# Autodesk Inventor assembly: rover-encoder-assembly
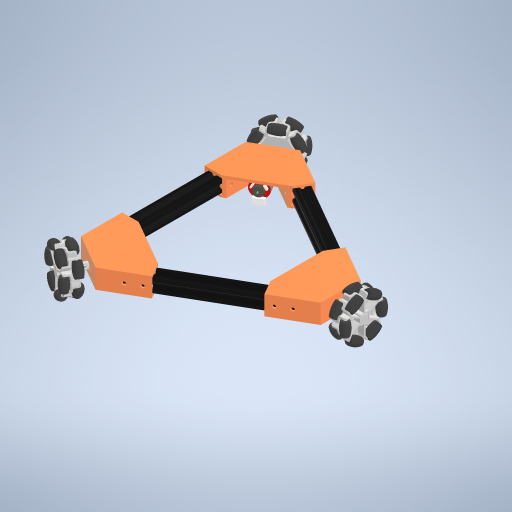
[picture p0: Inventor's stored thumbnail of the model, 512x512]
Saved by Autodesk Inventor 2024.2 (Build 282272000, 272)
## iProperties
Created: 2024-04-23
Part Number: rover-encoder-assembly
Document SubType Name: Assembly
Designer: Robin
Author: Robin
## Documents named in this file (6)
- C:\Users\Robin\OneDrive\Study\Current\Mechanical Design\Cad\fork-cad\rover-encoder-assembly.iam
- C:\Users\Robin\OneDrive\Study\Current\Mechanical Design\Cad\fork-cad\cornerBracket_Encoder.ipt
- C:\Users\Robin\OneDrive\Study\Current\Mechanical Design\Cad\fork-cad\2020aluminum_extrusion_black.ipt
- C:\Users\Robin\OneDrive\Study\Current\Mechanical Design\Cad\fork-cad\JGA25-370 DC12V350RPM\JGA25-370 DC12V350RPM.ipt
- C:\Users\Robin\OneDrive\Study\Current\Mechanical Design\Cad\fork-cad\wheel-assembly.iam
- C:\Users\Robin\OneDrive\Study\Current\Mechanical Design\Cad\fork-cad\holo-lock.ipt
## Components (15 placed, 5 different names)
1. cornerBracket_Encoder:1 — Mate:1, Mate:2, Mate:3, Mate:4, Mate:5, Mate:6, Mate:18, Mate:19, Mate:31
2. cornerBracket_Encoder:2 — Mate:10, Mate:11, Mate:12, Mate:13, Mate:14, Mate:15, Mate:17, Mate:20, Mate:33
3. cornerBracket_Encoder:3 — Mate:7, Mate:8, Mate:9, Mate:16, Mate:21, Mate:29
4. 2020aluminum_extrusion_black:1 — Mate:11, Mate:12, Mate:13
5. 2020aluminum_extrusion_black:2 — Mate:4, Mate:5, Mate:6, Mate:7, Mate:8, Mate:9
6. 2020aluminum_extrusion_black:3 — Mate:1, Mate:2, Mate:3, Mate:10, Mate:14, Mate:15
7. JGA25-370 DC12V350RPM:1 — Mate:17, Mate:20, Mate:32
8. JGA25-370 DC12V350RPM:2 — Mate:16, Mate:21, Mate:28
9. JGA25-370 DC12V350RPM:3 — Mate:18, Mate:19, Mate:30
10. wheel-assembly:1 [sub-assembly] — Mate:22, Mate:23, Flush:1
11. holo-lock:1 — Mate:22, Mate:23, Flush:1, Mate:32, Mate:33
12. wheel-assembly:4 [sub-assembly]
13. holo-lock:4 — Mate:30, Mate:31
14. wheel-assembly:5 [sub-assembly]
15. holo-lock:5 — Mate:28, Mate:29
## Relationships (36: Mate 33, Flush 3)
- Mate:1: cornerBracket_Encoder:1 ↔ 2020aluminum_extrusion_black:3
- Mate:2 (0.5 mm): cornerBracket_Encoder:1 ↔ 2020aluminum_extrusion_black:3
- Mate:3 (0.5 mm): cornerBracket_Encoder:1 ↔ 2020aluminum_extrusion_black:3
- Mate:4: cornerBracket_Encoder:1 ↔ 2020aluminum_extrusion_black:2
- Mate:5 (0.5 mm): cornerBracket_Encoder:1 ↔ 2020aluminum_extrusion_black:2
- Mate:6 (0.5 mm): cornerBracket_Encoder:1 ↔ 2020aluminum_extrusion_black:2
- Mate:7: cornerBracket_Encoder:3 ↔ 2020aluminum_extrusion_black:2
- Mate:8 (0.5 mm): cornerBracket_Encoder:3 ↔ 2020aluminum_extrusion_black:2
- Mate:9 (0.5 mm): cornerBracket_Encoder:3 ↔ 2020aluminum_extrusion_black:2
- Mate:10: cornerBracket_Encoder:2 ↔ 2020aluminum_extrusion_black:3
- Mate:11: cornerBracket_Encoder:2 ↔ 2020aluminum_extrusion_black:1
- Mate:12 (0.5 mm): cornerBracket_Encoder:2 ↔ 2020aluminum_extrusion_black:1
- Mate:13 (0.5 mm): cornerBracket_Encoder:2 ↔ 2020aluminum_extrusion_black:1
- Mate:14 (0.5 mm): cornerBracket_Encoder:2 ↔ 2020aluminum_extrusion_black:3
- Mate:15 (0.5 mm): cornerBracket_Encoder:2 ↔ 2020aluminum_extrusion_black:3
- Mate:16: cornerBracket_Encoder:3 ↔ JGA25-370 DC12V350RPM:2
- Mate:17: cornerBracket_Encoder:2 ↔ JGA25-370 DC12V350RPM:1
- Mate:18: cornerBracket_Encoder:1 ↔ JGA25-370 DC12V350RPM:3
- Mate:19: cornerBracket_Encoder:1 ↔ JGA25-370 DC12V350RPM:3
- Mate:20: cornerBracket_Encoder:2 ↔ JGA25-370 DC12V350RPM:1
- Mate:21: cornerBracket_Encoder:3 ↔ JGA25-370 DC12V350RPM:2
- Mate:22: wheel-assembly:1 ↔ holo-lock:1
- Mate:23: wheel-assembly:1 ↔ holo-lock:1
- Flush:1: wheel-assembly:1 ↔ holo-lock:1
- [Mate]: wheel-assembly:4 ↔ holo-lock:4
- [Mate]: wheel-assembly:4 ↔ holo-lock:4
- [Flush]: wheel-assembly:4 ↔ holo-lock:4
- [Mate]: wheel-assembly:5 ↔ holo-lock:5
- [Mate]: wheel-assembly:5 ↔ holo-lock:5
- [Flush]: wheel-assembly:5 ↔ holo-lock:5
- Mate:28: JGA25-370 DC12V350RPM:2 ↔ holo-lock:5
- Mate:29: cornerBracket_Encoder:3 ↔ holo-lock:5
- Mate:30: JGA25-370 DC12V350RPM:3 ↔ holo-lock:4
- Mate:31: cornerBracket_Encoder:1 ↔ holo-lock:4
- Mate:32: JGA25-370 DC12V350RPM:1 ↔ holo-lock:1
- Mate:33: cornerBracket_Encoder:2 ↔ holo-lock:1
## Named parameters: d24_d21 = 0 mm, d25_d22 = 0 mm, d26_d23 = 0 mm, d27_d21 = 0 mm, d28_d22 = 0 mm, d29_d23 = 0 mm
